# Autodesk Inventor assembly: matriz_biciclea
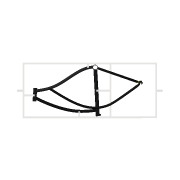
[picture p0: Inventor's stored thumbnail of the model, 180x180]
Saved by Autodesk Inventor 2021 (Build 250183000, 183)
## iProperties
Created: 2021-03-29
Part Number: matriz_biciclea
Document SubType Name: Assembly
Designer: j2seb
Author: j2seb
## Documents named in this file (7)
- E:\Documentos\Documentos\Michael_Rodriguez\ProyectoAPM\matriz_biciclea.iam
- E:\Documentos\Documentos\Michael_Rodriguez\Universidad_Nacional\Doceaba_matricula\Automatizacion\Proyecto\Proyecto_APM\02 Inventor\Esqueleto_estructura.ipt
- E:\Documentos\Documentos\Michael_Rodriguez\Universidad_Nacional\Doceaba_matricula\Automatizacion\Proyecto\Proyecto_APM\02 Inventor\Marco_Bicicleta\Frame\Estructura 1617045494032.iam
- E:\Documentos\Documentos\Michael_Rodriguez\Universidad_Nacional\Doceaba_matricula\Automatizacion\Proyecto\Proyecto_APM\02 Inventor\lamina_trasero.ipt
- E:\Documentos\Documentos\Michael_Rodriguez\Universidad_Nacional\Doceaba_matricula\Automatizacion\Proyecto\Proyecto_APM\02 Inventor\ajuste_silin.ipt
- E:\Documentos\Documentos\Michael_Rodriguez\ProyectoAPM\Pieza2.ipt
- E:\Documentos\Documentos\Michael_Rodriguez\ProyectoAPM\Pieza1.ipt
## Components (8 placed, 6 different names)
1. Esqueleto_estructura:1 — Coincidencia:2, Coincidencia:3, Coincidencia:4, Coincidencia:5, Coincidencia:6, Coincidencia:9, Coincidencia:10
2. Estructura 1617045494032:1 [sub-assembly] — Nivelación:5, Nivelación:6
3. lamina_trasero:1 — Coincidencia:7, Coincidencia:8, Nivelación:4
4. lamina_trasero:2 — Coincidencia:12, Coincidencia:14
5. ajuste_silin:1 — Nivelación:5
6. Pieza2:1 — Nivelación:6, Coincidencia:15, Coincidencia:16, Coincidencia:17, Coincidencia:18
7. Pieza1:1 — Coincidencia:15, Coincidencia:17
8. Pieza1:2 — Coincidencia:16, Coincidencia:18
## Relationships (21: Mate 17, Flush 4)
- Coincidencia:2 [Mate]: Esqueleto_estructura:1
- Coincidencia:3 [Mate]: Esqueleto_estructura:1
- Coincidencia:4 [Mate]: Esqueleto_estructura:1
- Coincidencia:5 [Mate]: Esqueleto_estructura:1
- Coincidencia:6 [Mate]: Esqueleto_estructura:1
- Nivelación:3 [Flush] (35 mm)
- Coincidencia:7 [Mate]: lamina_trasero:1
- Coincidencia:8 [Mate]: lamina_trasero:1
- Coincidencia:9 [Mate]: Esqueleto_estructura:1
- Coincidencia:10 [Mate]: Esqueleto_estructura:1
- Coincidencia:11 [Mate]
- Nivelación:4 [Flush] (55 mm): lamina_trasero:1
- Coincidencia:12 [Mate]: lamina_trasero:2
- Coincidencia:13 [Mate]
- Coincidencia:14 [Mate] (-55 mm): lamina_trasero:2
- Nivelación:5 [Flush]: Estructura 1617045494032:1 ↔ ajuste_silin:1
- Nivelación:6 [Flush] (-26 mm): Estructura 1617045494032:1 ↔ Pieza2:1
- Coincidencia:15 [Mate]: Pieza2:1 ↔ Pieza1:1
- Coincidencia:16 [Mate]: Pieza2:1 ↔ Pieza1:2
- Coincidencia:17 [Mate] (-312 mm): Pieza2:1 ↔ Pieza1:1
- Coincidencia:18 [Mate] (-312 mm): Pieza2:1 ↔ Pieza1:2
